# Autodesk Inventor assembly: 2AM-17-A-2200 - slider outside
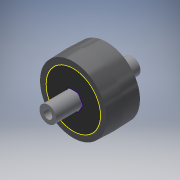
[picture p0: Inventor's stored thumbnail of the model, 180x180]
Saved by Autodesk Inventor 2017 (Build 210142000, 142)
## iProperties
Created: 2017-12-27
Part Number: 2AM-17-A-2200 - slider outside
Document SubType Name: Assembly
Designer: Micah
Author: Micah
## Documents named in this file (3)
- C:\Users\Micah\Desktop\inventor\CADathon-2017\2AM-17-A-0200 - Smokestack Elevator\2AM-17-A-2200 - slider outside.iam
- C:\Users\Micah\Desktop\inventor\CADathon-2017\2AM-17-A-0200 - Smokestack Elevator\2AM-17-A-3200 - wheels for outside slider.iam
- C:\Users\Micah\Desktop\inventor\CADathon-2017\2AM-17-A-0200 - Smokestack Elevator\2AM-17-P-2202 - tube shaft.ipt
## Components (2 placed, 2 different names)
1. 2AM-17-A-3200 - wheels for outside slider:2 [sub-assembly] — Rotational:1
2. 2AM-17-P-2202 - tube shaft:1 — Rotational:1
## Relationships (1: RevoluteJoint 1)
- Rotational:1 [RevoluteJoint] (-19.05 mm): 2AM-17-A-3200 - wheels for outside slider:2 ↔ 2AM-17-P-2202 - tube shaft:1
